# Autodesk Inventor assembly: ASSEMBLY_Main
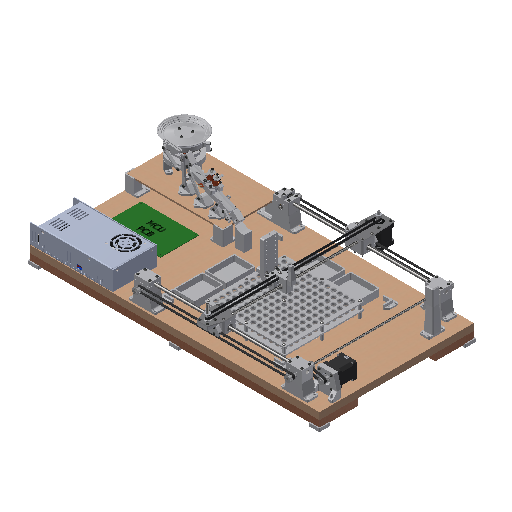
[picture p0: Inventor's stored thumbnail of the model, 512x512]
Saved by Autodesk Inventor 2026.1 (Build 301233000, 233)
## iProperties
Created: 2018-06-14
Part Number: ASSEMBLY_Main
Document SubType Name: Assembly
Designer: Andrzej
Author: Andrzej
## Documents named in this file (16)
- C:\Users\Andrzej\OneDrive\_DRIVE_SYNCH_FILES\__ BYTECHLAB PROJECTS\MLTDIS - SMD Parts Sorting Machine\MCAD\1_REV1\ASSEMBLY_MAIN_REVA\ASSEMBLY_Main.iam
- C:\Users\Andrzej\OneDrive\_DRIVE_SYNCH_FILES\__ BYTECHLAB PROJECTS\MLTDIS - SMD Parts Sorting Machine\MCAD\1_REV1\ASSEMBLY_BOWL_FEEDER_REVA\ASSEMBLY_MAIN_REVA\ASSEMBLY_Main_Bowl_Feeder.iam
- C:\Users\Andrzej\OneDrive\_DRIVE_SYNCH_FILES\__ BYTECHLAB PROJECTS\MLTDIS - SMD Parts Sorting Machine\MCAD\1_REV1\ASSEMBLY_MEASUREMENT_RAIL_REVA\ASSEMBLY_MAIN_REVA\ASSEMBLY_Main_Measurement_Rail.iam
- C:\Users\Andrzej\OneDrive\_DRIVE_SYNCH_FILES\__ BYTECHLAB PROJECTS\MLTDIS - SMD Parts Sorting Machine\MCAD\1_REV1\ASSEMBLY_MAIN_REVA\CNCM_WOOD_18mm_Base_plate.ipt
- C:\Users\Andrzej\OneDrive\_DRIVE_SYNCH_FILES\__ BYTECHLAB PROJECTS\MLTDIS - SMD Parts Sorting Machine\MCAD\1_REV1\ASSEMBLY_TEST_TUBE_ARRAY_REVA\ASSEMBLY_Main_Test_tube_array.iam
- C:\Users\Andrzej\OneDrive\_DRIVE_SYNCH_FILES\__ BYTECHLAB PROJECTS\MLTDIS - SMD Parts Sorting Machine\MCAD\1_REV1\ASSEMBLY_XY_AXIS_REVA\ASSEMBLY_Main_XY_Axis.iam
- C:\Users\Andrzej\OneDrive\_DRIVE_SYNCH_FILES\__ BYTECHLAB PROJECTS\MLTDIS - SMD Parts Sorting Machine\MCAD\1_REV1\ASSEMBLY_MAIN_REVA\CNCM_WOOD_4mm_Sorting_line_base_plate.ipt
- C:\Users\Andrzej\OneDrive\_DRIVE_SYNCH_FILES\__ BYTECHLAB PROJECTS\MLTDIS - SMD Parts Sorting Machine\MCAD\1_REV1\ASSEMBLY_MAIN_REVA\CNCM_WOOD_18mm_Base_plate_reinforcement.ipt
- C:\Users\Andrzej\OneDrive\_DRIVE_SYNCH_FILES\__ BYTECHLAB PROJECTS\MLTDIS - SMD Parts Sorting Machine\MCAD\1_REV1\ASSEMBLY_MAIN_REVA\3DP_PLA_Base_plate_corner_leg.ipt
- C:\Users\Andrzej\OneDrive\_DRIVE_SYNCH_FILES\__ BYTECHLAB PROJECTS\MLTDIS - SMD Parts Sorting Machine\MCAD\1_REV1\ASSEMBLY_MAIN_REVA\3DP_PLA_Base_plate_side_leg.ipt
- C:\Users\Andrzej\OneDrive\_DRIVE_SYNCH_FILES\__ BYTECHLAB PROJECTS\MLTDIS - SMD Parts Sorting Machine\MCAD\1_REV1\ASSEMBLY_MAIN_REVA\3DP_PLA_Base_plate_wire_harness_mount.ipt
- C:\Users\Andrzej\OneDrive\_DRIVE_SYNCH_FILES\__ BYTECHLAB PROJECTS\MLTDIS - SMD Parts Sorting Machine\MCAD\1_REV1\__COTS_PARTS\COTS_GENERIC_12V_PSU\COTS_GENERIC_12V_PSU.iam
- C:\Users\Andrzej\OneDrive\_DRIVE_SYNCH_FILES\__ BYTECHLAB PROJECTS\MLTDIS - SMD Parts Sorting Machine\MCAD\1_REV1\ASSEMBLY_MAIN_REVA\3DP_PLA_Sorting_line_base_plate_standoff.ipt
- C:\Users\Andrzej\OneDrive\_DRIVE_SYNCH_FILES\__ BYTECHLAB PROJECTS\MLTDIS - SMD Parts Sorting Machine\MCAD\1_REV1\ASSEMBLY_MAIN_REVA\ASSEMBLY_Controller_PCB.ipt
- C:\Users\Andrzej\OneDrive\_DRIVE_SYNCH_FILES\__ BYTECHLAB PROJECTS\MLTDIS - SMD Parts Sorting Machine\MCAD\1_REV1\ASSEMBLY_MAIN_REVA\3DP_PLA_Tray_for_unknown_parts.ipt
- C:\Users\Andrzej\OneDrive\_DRIVE_SYNCH_FILES\__ BYTECHLAB PROJECTS\MLTDIS - SMD Parts Sorting Machine\MCAD\1_REV1\ASSEMBLY_MAIN_REVA\3DP_PLA_Pick_up_tray.ipt
## Components (26 placed, 15 different names)
1. ASSEMBLY_Main_Bowl_Feeder:1 [sub-assembly] — Mate:29
2. ASSEMBLY_Main_Measurement_Rail:1 [sub-assembly] — Mate:12
3. CNCM_WOOD_18mm_Base_plate:1 — Mate:3, Mate:32, Mate:33, Flush:6, Flush:7, Flush:8, Flush:9, Mate:34, Flush:10, Flush:11, Mate:51, Flush:14, Mate:52, Flush:15, Flush:16, Mate:53, Mate:54, Mate:55, Mate:56, Flush:17, Flush:18, Mate:66, Mate:67, Mate:69, Mate:70, Mate:71, Mate:72
4. ASSEMBLY_Main_Test_tube_array:1 [sub-assembly] — Mate:3
5. CNCM_WOOD_4mm_Sorting_line_base_plate:1 — Mate:12, Mate:29, Mate:57, Mate:58, Mate:59, Mate:60, Mate:61, Mate:62, Mate:63, Mate:64, Mate:65
6. CNCM_WOOD_18mm_Base_plate_reinforcement:1 — Mate:33, Flush:6, Flush:7, Mate:37, Mate:39, Mate:40, Mate:46, Mate:47, Mate:48, Mate:49, Mate:50, Flush:12
7. CNCM_WOOD_18mm_Base_plate_reinforcement:2 — Mate:32, Flush:8, Flush:9, Mate:35, Mate:36, Mate:38, Mate:41, Mate:42, Mate:43, Mate:44, Mate:45
8. ASSEMBLY_Main_XY_Axis:1 [sub-assembly] — Mate:34, Flush:10, Flush:11, Mate:68
9. 3DP_PLA_Base_plate_corner_leg:1 — Mate:35, Mate:41, Mate:42
10. 3DP_PLA_Base_plate_side_leg:1 — Mate:40, Mate:50, Flush:12, Flush:13
11. 3DP_PLA_Base_plate_corner_leg:2 — Mate:37, Mate:48, Mate:49
12. 3DP_PLA_Base_plate_side_leg:2 — Mate:38, Mate:43, Flush:13
13. 3DP_PLA_Base_plate_corner_leg:3 — Mate:39, Mate:46, Mate:47
14. 3DP_PLA_Base_plate_corner_leg:4 — Mate:36, Mate:44, Mate:45
15. 3DP_PLA_Base_plate_wire_harness_mount:1 — Mate:51, Flush:14
16. COTS_GENERIC_12V_PSU:1 [sub-assembly] — Mate:52, Flush:15, Flush:16
17. 3DP_PLA_Sorting_line_base_plate_standoff:1 — Mate:55, Mate:62, Mate:63
18. 3DP_PLA_Sorting_line_base_plate_standoff:2 — Mate:54, Mate:60, Mate:61, Flush:17, Flush:18
19. 3DP_PLA_Sorting_line_base_plate_standoff:3 — Mate:56, Mate:64, Mate:65
20. 3DP_PLA_Sorting_line_base_plate_standoff:4 — Mate:53, Mate:57, Mate:58, Mate:59
21. ASSEMBLY_Controller_PCB:1 — Mate:66
22. 3DP_PLA_Tray_for_unknown_parts:1 — Mate:67, Mate:68, Flush:19
23. 3DP_PLA_Pick_up_tray:1 — Mate:69
24. 3DP_PLA_Tray_for_unknown_parts:2 — Mate:71, Flush:20
25. 3DP_PLA_Tray_for_unknown_parts:3 — Mate:70, Flush:19
26. 3DP_PLA_Tray_for_unknown_parts:4 — Mate:72, Flush:20
## Relationships (59: Mate 44, Flush 15)
- Mate:3: CNCM_WOOD_18mm_Base_plate:1 ↔ ASSEMBLY_Main_Test_tube_array:1
- Mate:12: ASSEMBLY_Main_Measurement_Rail:1 ↔ CNCM_WOOD_4mm_Sorting_line_base_plate:1
- Mate:29: ASSEMBLY_Main_Bowl_Feeder:1 ↔ CNCM_WOOD_4mm_Sorting_line_base_plate:1
- Mate:32: CNCM_WOOD_18mm_Base_plate:1 ↔ CNCM_WOOD_18mm_Base_plate_reinforcement:2
- Mate:33: CNCM_WOOD_18mm_Base_plate:1 ↔ CNCM_WOOD_18mm_Base_plate_reinforcement:1
- Flush:6: CNCM_WOOD_18mm_Base_plate:1 ↔ CNCM_WOOD_18mm_Base_plate_reinforcement:1
- Flush:7: CNCM_WOOD_18mm_Base_plate:1 ↔ CNCM_WOOD_18mm_Base_plate_reinforcement:1
- Flush:8: CNCM_WOOD_18mm_Base_plate:1 ↔ CNCM_WOOD_18mm_Base_plate_reinforcement:2
- Flush:9: CNCM_WOOD_18mm_Base_plate:1 ↔ CNCM_WOOD_18mm_Base_plate_reinforcement:2
- Mate:34: CNCM_WOOD_18mm_Base_plate:1 ↔ ASSEMBLY_Main_XY_Axis:1
- Flush:10 (5 mm): CNCM_WOOD_18mm_Base_plate:1 ↔ ASSEMBLY_Main_XY_Axis:1
- Flush:11 (3.1 mm): CNCM_WOOD_18mm_Base_plate:1 ↔ ASSEMBLY_Main_XY_Axis:1
- Mate:35: CNCM_WOOD_18mm_Base_plate_reinforcement:2 ↔ 3DP_PLA_Base_plate_corner_leg:1
- Mate:36: CNCM_WOOD_18mm_Base_plate_reinforcement:2 ↔ 3DP_PLA_Base_plate_corner_leg:4
- Mate:37: CNCM_WOOD_18mm_Base_plate_reinforcement:1 ↔ 3DP_PLA_Base_plate_corner_leg:2
- Mate:38: CNCM_WOOD_18mm_Base_plate_reinforcement:2 ↔ 3DP_PLA_Base_plate_side_leg:2
- Mate:39: CNCM_WOOD_18mm_Base_plate_reinforcement:1 ↔ 3DP_PLA_Base_plate_corner_leg:3
- Mate:40: CNCM_WOOD_18mm_Base_plate_reinforcement:1 ↔ 3DP_PLA_Base_plate_side_leg:1
- Mate:41: CNCM_WOOD_18mm_Base_plate_reinforcement:2 ↔ 3DP_PLA_Base_plate_corner_leg:1
- Mate:42: CNCM_WOOD_18mm_Base_plate_reinforcement:2 ↔ 3DP_PLA_Base_plate_corner_leg:1
- Mate:43: CNCM_WOOD_18mm_Base_plate_reinforcement:2 ↔ 3DP_PLA_Base_plate_side_leg:2
- Mate:44: CNCM_WOOD_18mm_Base_plate_reinforcement:2 ↔ 3DP_PLA_Base_plate_corner_leg:4
- Mate:45: CNCM_WOOD_18mm_Base_plate_reinforcement:2 ↔ 3DP_PLA_Base_plate_corner_leg:4
- Mate:46: CNCM_WOOD_18mm_Base_plate_reinforcement:1 ↔ 3DP_PLA_Base_plate_corner_leg:3
- Mate:47: CNCM_WOOD_18mm_Base_plate_reinforcement:1 ↔ 3DP_PLA_Base_plate_corner_leg:3
- Mate:48: CNCM_WOOD_18mm_Base_plate_reinforcement:1 ↔ 3DP_PLA_Base_plate_corner_leg:2
- Mate:49: CNCM_WOOD_18mm_Base_plate_reinforcement:1 ↔ 3DP_PLA_Base_plate_corner_leg:2
- Mate:50: CNCM_WOOD_18mm_Base_plate_reinforcement:1 ↔ 3DP_PLA_Base_plate_side_leg:1
- Flush:12 (362.5 mm): CNCM_WOOD_18mm_Base_plate_reinforcement:1 ↔ 3DP_PLA_Base_plate_side_leg:1
- Flush:13: 3DP_PLA_Base_plate_side_leg:1 ↔ 3DP_PLA_Base_plate_side_leg:2
- Mate:51: CNCM_WOOD_18mm_Base_plate:1 ↔ 3DP_PLA_Base_plate_wire_harness_mount:1
- Flush:14 (20 mm): CNCM_WOOD_18mm_Base_plate:1 ↔ 3DP_PLA_Base_plate_wire_harness_mount:1
- Mate:52: CNCM_WOOD_18mm_Base_plate:1 ↔ COTS_GENERIC_12V_PSU:1
- Flush:15: CNCM_WOOD_18mm_Base_plate:1 ↔ COTS_GENERIC_12V_PSU:1
- Flush:16: CNCM_WOOD_18mm_Base_plate:1 ↔ COTS_GENERIC_12V_PSU:1
- Mate:53: CNCM_WOOD_18mm_Base_plate:1 ↔ 3DP_PLA_Sorting_line_base_plate_standoff:4
- Mate:54: CNCM_WOOD_18mm_Base_plate:1 ↔ 3DP_PLA_Sorting_line_base_plate_standoff:2
- Mate:55: CNCM_WOOD_18mm_Base_plate:1 ↔ 3DP_PLA_Sorting_line_base_plate_standoff:1
- Mate:56: CNCM_WOOD_18mm_Base_plate:1 ↔ 3DP_PLA_Sorting_line_base_plate_standoff:3
- Mate:57: CNCM_WOOD_4mm_Sorting_line_base_plate:1 ↔ 3DP_PLA_Sorting_line_base_plate_standoff:4
- Mate:58: CNCM_WOOD_4mm_Sorting_line_base_plate:1 ↔ 3DP_PLA_Sorting_line_base_plate_standoff:4
- Mate:59: CNCM_WOOD_4mm_Sorting_line_base_plate:1 ↔ 3DP_PLA_Sorting_line_base_plate_standoff:4
- Mate:60: CNCM_WOOD_4mm_Sorting_line_base_plate:1 ↔ 3DP_PLA_Sorting_line_base_plate_standoff:2
- Mate:61: CNCM_WOOD_4mm_Sorting_line_base_plate:1 ↔ 3DP_PLA_Sorting_line_base_plate_standoff:2
- Mate:62: CNCM_WOOD_4mm_Sorting_line_base_plate:1 ↔ 3DP_PLA_Sorting_line_base_plate_standoff:1
- Mate:63: CNCM_WOOD_4mm_Sorting_line_base_plate:1 ↔ 3DP_PLA_Sorting_line_base_plate_standoff:1
- Mate:64: CNCM_WOOD_4mm_Sorting_line_base_plate:1 ↔ 3DP_PLA_Sorting_line_base_plate_standoff:3
- Mate:65: CNCM_WOOD_4mm_Sorting_line_base_plate:1 ↔ 3DP_PLA_Sorting_line_base_plate_standoff:3
- Flush:17: CNCM_WOOD_18mm_Base_plate:1 ↔ 3DP_PLA_Sorting_line_base_plate_standoff:2
- Flush:18: CNCM_WOOD_18mm_Base_plate:1 ↔ 3DP_PLA_Sorting_line_base_plate_standoff:2
- Mate:66 (10 mm): CNCM_WOOD_18mm_Base_plate:1 ↔ ASSEMBLY_Controller_PCB:1
- Mate:67: CNCM_WOOD_18mm_Base_plate:1 ↔ 3DP_PLA_Tray_for_unknown_parts:1
- Mate:68 (5 mm): ASSEMBLY_Main_XY_Axis:1 ↔ 3DP_PLA_Tray_for_unknown_parts:1
- Mate:69: CNCM_WOOD_18mm_Base_plate:1 ↔ 3DP_PLA_Pick_up_tray:1
- Mate:70: CNCM_WOOD_18mm_Base_plate:1 ↔ 3DP_PLA_Tray_for_unknown_parts:3
- Mate:71: CNCM_WOOD_18mm_Base_plate:1 ↔ 3DP_PLA_Tray_for_unknown_parts:2
- Flush:19: 3DP_PLA_Tray_for_unknown_parts:1 ↔ 3DP_PLA_Tray_for_unknown_parts:3
- Mate:72: CNCM_WOOD_18mm_Base_plate:1 ↔ 3DP_PLA_Tray_for_unknown_parts:4
- Flush:20: 3DP_PLA_Tray_for_unknown_parts:2 ↔ 3DP_PLA_Tray_for_unknown_parts:4
